# Autodesk Inventor assembly: Arm System
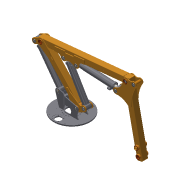
[picture p0: Inventor's stored thumbnail of the model, 180x180]
Saved by Autodesk Inventor 2022 Beta2 (Build 260130000, 130) ContinuousBuild 0
## iProperties
Shininess: 64.0
Length Units: 11269
Angle Units: 11279
Time Units: 11290
Mass Units: 11283
Length Display Precision: 3
Angle Display Precision: 2
Created: 2002-06-11
Part Number: Arm System
Document SubType Name: Assembly
Designer: Joe M
Engineer: Joe M
Density: 0.0
Volumn: 0.0
Area: 0.0
PropertySet Name: Model Information
Control State: 0
Master: False
Checked Out: False
Author: Joe M
## Documents named in this file (6)
- C:\Autodesk Inventor 2021 Intro Practice Files\BOM\Arm System.iam
- C:\Autodesk Inventor 2021 Intro Practice Files\BOM\Cylinder.iam
- C:\Autodesk Inventor 2021 Intro Practice Files\BOM\Lower Arm-N.iam
- C:\Autodesk Inventor 2021 Intro Practice Files\BOM\Middle Arm-N.iam
- C:\Autodesk Inventor 2021 Intro Practice Files\BOM\Armbracket-Base.iam
- C:\Autodesk Inventor 2021 Intro Practice Files\BOM\Top Arm-N.iam
## Components (7 placed, 5 different names)
1. Armbracket-Base:1 [sub-assembly] — Mate:4, Mate:5, Mate:6, Mate:8
2. Lower Arm-N:1 [sub-assembly] — Mate:6, Mate:8, Mate:9, Mate:10, Mate:12, Insert:1
3. Middle Arm-N:1 [sub-assembly] — Mate:10, Mate:12, Mate:17, Mate:18, Insert:2, Mate:24
4. Top Arm-N:1 [sub-assembly] — Mate:17, Mate:18, Mate:22
5. Cylinder:1 [sub-assembly] — Mate:4, Mate:5, Mate:9
6. Cylinder:2 [sub-assembly] — Insert:1, Mate:24
7. Cylinder:3 [sub-assembly] — Insert:2, Mate:22
## Relationships (13: Mate 11, Insert 2)
- Mate:4: Armbracket-Base:1 ↔ Cylinder:1
- Mate:5 (0.25 mm): Armbracket-Base:1 ↔ Cylinder:1
- Mate:6: Armbracket-Base:1 ↔ Lower Arm-N:1
- Mate:8 (2.25 mm): Armbracket-Base:1 ↔ Lower Arm-N:1
- Mate:9: Lower Arm-N:1 ↔ Cylinder:1
- Mate:10: Lower Arm-N:1 ↔ Middle Arm-N:1
- Mate:12: Lower Arm-N:1 ↔ Middle Arm-N:1
- Mate:17: Middle Arm-N:1 ↔ Top Arm-N:1
- Mate:18: Middle Arm-N:1 ↔ Top Arm-N:1
- Insert:1: Lower Arm-N:1 ↔ Cylinder:2
- Insert:2: Middle Arm-N:1 ↔ Cylinder:3
- Mate:22: Top Arm-N:1 ↔ Cylinder:3
- Mate:24: Middle Arm-N:1 ↔ Cylinder:2
